# Autodesk Inventor assembly: Assembly_Opentrons_Autofocus_v0
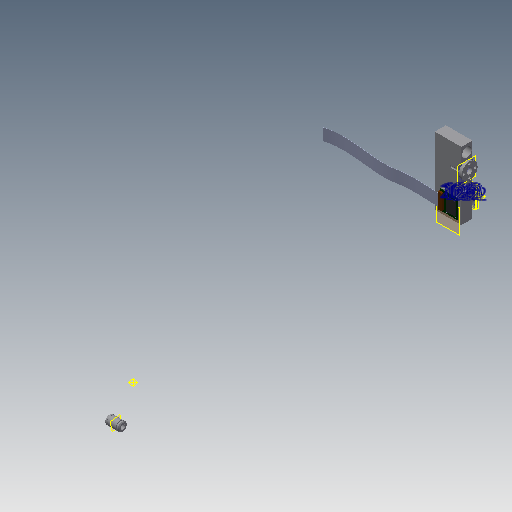
[picture p0: Inventor's stored thumbnail of the model, 512x512]
Saved by Autodesk Inventor 2019.4 (Build 234330000, 330)
## iProperties
Created: 2020-10-23
Part Number: Assembly_Opentrons_Autofocus_v0
Document SubType Name: Assembly
Designer: diederichbenedict
Author: diederichbenedict
## Documents named in this file (9)
- C:\Users\diederichbenedict\Dropbox\Dokumente\Promotion\PROJECTS\OPENTRONS\INVENTOR\Assembly_Opentrons_Autofocus_v0.iam
- C:\Users\diederichbenedict\Dropbox\Dokumente\Promotion\PROJECTS\OPENTRONS\INVENTOR\00_CCTV_Fisheye_Starlight_f2.8mm_Fno_1.4.ipt
- C:\Users\diederichbenedict\Dropbox\Dokumente\Promotion\PROJECTS\OPENTRONS\INVENTOR\00_Ringmagnet_25mm.ipt
- C:\Users\diederichbenedict\Dropbox\Dokumente\Promotion\PROJECTS\OPENTRONS\INVENTOR\01_Autofocus_CCTV12mm_spring_1.ipt
- C:\Users\diederichbenedict\Dropbox\Dokumente\Promotion\PROJECTS\OPENTRONS\INVENTOR\00_RasPi_Camera.ipt
- C:\Users\diederichbenedict\Dropbox\Dokumente\Promotion\PROJECTS\OPENTRONS\INVENTOR\01_Autofocus_Magnet_holder_v0.ipt
- C:\Users\diederichbenedict\Dropbox\Dokumente\Promotion\PROJECTS\OPENTRONS\INVENTOR\01_Slide_camera_x_v0.ipt
- C:\Users\diederichbenedict\Dropbox\Dokumente\Promotion\PROJECTS\OPENTRONS\INVENTOR\00_IGUS_Drylin_RJ4JP-01-06.ipt
- C:\Users\diederichbenedict\Dropbox\Dokumente\Promotion\PROJECTS\OPENTRONS\INVENTOR\00_spindel_slide.ipt
## Components (12 placed, 8 different names)
1. 00_CCTV_Fisheye_Starlight_f2.8mm_Fno_1.4:1 — Mate:1, Mate:2, Mate:3, Flush:1
2. 00_Ringmagnet_25mm:1 — Insert:1, Angle:1, Insert:3, Flush:1, Flush:2, Flush:3
3. 00_Ringmagnet_25mm:2 — Insert:1, Insert:2
4. 00_Ringmagnet_25mm:3 — Insert:2, Mate:1
5. 01_Autofocus_CCTV12mm_spring_1:1 — Insert:3, Insert:4
6. 01_Autofocus_CCTV12mm_spring_1:2 — Insert:4
7. 00_RasPi_Camera:1 — Mate:2, Angle:2, Mate:3
8. 01_Autofocus_Magnet_holder_v0:1 — Flush:2, Flush:3
9. 00_IGUS_Drylin_RJ4JP-01-06:1
10. 00_IGUS_Drylin_RJ4JP-01-06:2
11. 00_spindel_slide:1 — Insert:5
12. 01_Slide_camera_x_v0:1 — Insert:5
## Relationships (14: Insert 5, Flush 4, Mate 3, Angle 2)
- Insert:1: 00_Ringmagnet_25mm:1 ↔ 00_Ringmagnet_25mm:2
- Insert:2: 00_Ringmagnet_25mm:2 ↔ 00_Ringmagnet_25mm:3
- Mate:1: 00_CCTV_Fisheye_Starlight_f2.8mm_Fno_1.4:1 ↔ 00_Ringmagnet_25mm:3
- Angle:1 (0 deg): 00_Ringmagnet_25mm:1
- Insert:3: 00_Ringmagnet_25mm:1 ↔ 01_Autofocus_CCTV12mm_spring_1:1
- Insert:4: 01_Autofocus_CCTV12mm_spring_1:1 ↔ 01_Autofocus_CCTV12mm_spring_1:2
- Mate:2: 00_CCTV_Fisheye_Starlight_f2.8mm_Fno_1.4:1 ↔ 00_RasPi_Camera:1
- Angle:2 (0 deg): 00_RasPi_Camera:1
- Mate:3 (10 mm): 00_CCTV_Fisheye_Starlight_f2.8mm_Fno_1.4:1 ↔ 00_RasPi_Camera:1
- Flush:1 (-2 mm): 00_CCTV_Fisheye_Starlight_f2.8mm_Fno_1.4:1 ↔ 00_Ringmagnet_25mm:1
- Flush:2: 00_Ringmagnet_25mm:1 ↔ 01_Autofocus_Magnet_holder_v0:1
- Flush:3: 00_Ringmagnet_25mm:1 ↔ 01_Autofocus_Magnet_holder_v0:1
- [Flush]: 01_Autofocus_Magnet_holder_v0:1 ↔ 01_Slide_camera_x_v0:1
- Insert:5: 00_spindel_slide:1 ↔ 01_Slide_camera_x_v0:1
## Named parameters: d13_d8 = 0 mm
